# Autodesk Inventor assembly: FirstAssembly
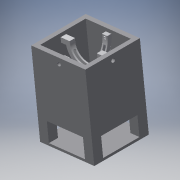
[picture p0: Inventor's stored thumbnail of the model, 180x180]
Saved by Autodesk Inventor 2017 (Build 210142000, 142)
## iProperties
Created: 2017-02-25
Part Number: FirstAssembly
Document SubType Name: Assembly
Designer: aribu
Author: aribu
## Documents named in this file (5)
- C:\Users\aribu\Dropbox\Kettering\CE-490 CE Capstone\GitHub\Hardware\Inventor Files\V2\FirstAssembly.iam
- C:\Users\aribu\Dropbox\Kettering\CE-490 CE Capstone\GitHub\Hardware\Inventor Files\V2\BottomCircleArm.ipt
- C:\Users\aribu\Dropbox\Kettering\CE-490 CE Capstone\GitHub\Hardware\Inventor Files\V2\Box.ipt
- C:\Users\aribu\Dropbox\Kettering\CE-490 CE Capstone\GitHub\Hardware\Inventor Files\V2\FalseFloor.ipt
- C:\Users\aribu\Dropbox\Kettering\CE-490 CE Capstone\GitHub\Hardware\Inventor Files\V2\TopCircleArm.ipt
## Components (4 placed, 4 different names)
1. BottomCircleArm:1 — Rotational:2
2. Box:1 — Mate:1, Flush:1, Flush:2, Rotational:1, Rotational:2
3. FalseFloor:1 — Mate:1, Flush:1, Flush:2
4. TopCircleArm:1 — Rotational:1
## Relationships (5: Flush 2, RevoluteJoint 2, Mate 1)
- Mate:1: Box:1 ↔ FalseFloor:1
- Flush:1: Box:1 ↔ FalseFloor:1
- Flush:2: Box:1 ↔ FalseFloor:1
- Rotational:1 [RevoluteJoint]: Box:1 ↔ TopCircleArm:1
- Rotational:2 [RevoluteJoint]: BottomCircleArm:1 ↔ Box:1
